# Autodesk Inventor assembly: Horn_Spacer_16
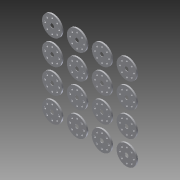
[picture p0: Inventor's stored thumbnail of the model, 180x180]
Saved by Autodesk Inventor 2013 (Build 170138000, 138)
## iProperties
Created: 2014-04-21
Part Number: Horn_Spacer_16
Document SubType Name: Assembly
Designer: andou
Author: andou
## Documents named in this file (2)
- C:\Users\andou\Documents\GitHub\Robotics-Project\design\RoboticsProject\project_4\cnc_data\Horn_Spacer_16.iam
- C:\Users\andou\Documents\GitHub\Robotics-Project\design\RoboticsProject\project_4\cnc_data\Leg_Horn_Spacer.ipt
## Components (16 placed, 1 different names)
1. Leg_Horn_Spacer:1
2. Leg_Horn_Spacer:2
3. Leg_Horn_Spacer:3
4. Leg_Horn_Spacer:4
5. Leg_Horn_Spacer:5
6. Leg_Horn_Spacer:6
7. Leg_Horn_Spacer:7
8. Leg_Horn_Spacer:8
9. Leg_Horn_Spacer:9
10. Leg_Horn_Spacer:10
11. Leg_Horn_Spacer:11
12. Leg_Horn_Spacer:12
13. Leg_Horn_Spacer:13
14. Leg_Horn_Spacer:14
15. Leg_Horn_Spacer:15
16. Leg_Horn_Spacer:16
## Component patterns: (16 elements, first: Leg_Horn_Spacer:1)
